# Autodesk Inventor assembly: OpenMV&Ping
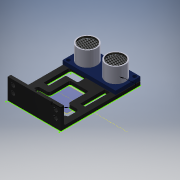
[picture p0: Inventor's stored thumbnail of the model, 180x180]
Saved by Autodesk Inventor 2018 (Build 220112000, 112)
## iProperties
Created: 2018-11-27
Part Number: OpenMV&Ping
Material: 一般
Document SubType Name: Assembly
Designer: shun2
Author: shun2
## Documents named in this file (3)
- C:\Users\shun2\OneDrive\おそらく最新版(2018.7.31)\OpenMV&Ping.iam
- C:\Users\shun2\OneDrive\おそらく最新版(2018.7.31)\OpenMV&Ping.ipt
- C:\Users\shun2\OneDrive\おそらく最新版(2018.7.31)\ping.ipt
## Components (2 placed, 2 different names)
1. OpenMV&Ping:1 — メイト:1, メイト:2, メイト:3
2. ping:1 — メイト:1, メイト:2, メイト:3
## Relationships (3: Mate 3)
- メイト:1 [Mate] (0.5 mm): OpenMV&Ping:1 ↔ ping:1
- メイト:2 [Mate]: OpenMV&Ping:1 ↔ ping:1
- メイト:3 [Mate]: OpenMV&Ping:1 ↔ ping:1
